# Autodesk Inventor assembly: rawPanel
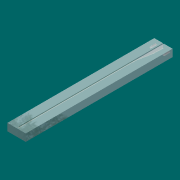
[picture p0: Inventor's stored thumbnail of the model, 180x180]
Saved by Autodesk Inventor 2016 SP1 (Build 200210100, 210)
## iProperties
Created: 2016-02-15
Part Number: rawPanel
Document SubType Name: Assembly
Designer: sawai
Author: sawai
## Documents named in this file (3)
- C:\Users\sawai\OneDrive\projects\scintillatorPanel\rawPanel.iam
- C:\Users\sawai\OneDrive\projects\scintillatorPanel\fiber.ipt
- C:\Users\sawai\OneDrive\projects\scintillatorPanel\fingerPanel.ipt
## Components (2 placed, 2 different names)
1. fiber:1 — Flush:1, Mate:1, Mate:2
2. fingerPanel:1 — Flush:1, Mate:1, Mate:2
## Relationships (3: Mate 2, Flush 1)
- Flush:1: fiber:1 ↔ fingerPanel:1
- Mate:1: fiber:1 ↔ fingerPanel:1
- Mate:2: fiber:1 ↔ fingerPanel:1
